# Autodesk Inventor assembly: base mg996r 3mm frame top
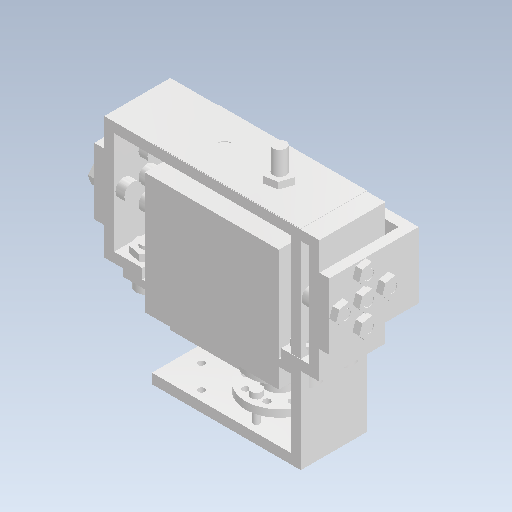
[picture p0: Inventor's stored thumbnail of the model, 512x512]
Saved by Autodesk Inventor 2021.4 (Build 254397000, 397)
## iProperties
Created: 2022-07-09
Part Number: base mg996r 3mm frame top
Document SubType Name: Assembly
Designer: isamu
Author: isamu
## Documents named in this file (5)
- D:\personal_projects\robot\inventor\2021\base mg996r 3mm frame top.iam
- D:\personal_projects\robot\exports\frames\servo frame part 3.ipt
- D:\personal_projects\robot\exports\screws\m3x8.ipt
- D:\personal_projects\robot\exports\screws\m3 nuts.ipt
- D:\personal_projects\robot\inventor\2021\base mg996r 3mm frame with axis.iam
## Components (22 placed, 4 different names)
1. servo frame part 3:1 — Mate:1, Mate:2, Mate:3, Insert:16, Insert:17, Insert:18, Insert:19, Insert:20, Insert:21, Insert:22, Insert:23, Insert:24, Insert:25
2. m3x8:1 — Insert:3
3. m3x8:2 — Insert:5
4. m3x8:3 — Insert:6
5. m3x8:4 — Insert:9
6. m3x8:5 — Insert:7
7. m3x8:6 — Insert:8
8. m3x8:7 — Insert:10
9. m3x8:9 — Insert:1
10. m3x8:11 — Insert:2
11. m3x8:12 — Insert:4
12. m3 nuts:1 — Insert:23
13. m3 nuts:2 — Insert:19
14. m3 nuts:3 — Insert:18
15. m3 nuts:4 — Insert:17
16. m3 nuts:5 — Insert:16
17. m3 nuts:6 — Insert:20
18. m3 nuts:7 — Insert:22
19. m3 nuts:8 — Insert:24
20. m3 nuts:9 — Insert:25
21. m3 nuts:10 — Insert:21
22. base mg996r 3mm frame with axis:1 [sub-assembly] — Mate:1, Mate:2, Mate:3, Insert:1, Insert:2, Insert:3, Insert:4, Insert:5, Insert:6, Insert:7, Insert:8, Insert:9, Insert:10
## Relationships (23: Insert 20, Mate 3)
- Mate:1: servo frame part 3:1 ↔ base mg996r 3mm frame with axis:1
- Mate:2: servo frame part 3:1 ↔ base mg996r 3mm frame with axis:1
- Mate:3: servo frame part 3:1 ↔ base mg996r 3mm frame with axis:1
- Insert:1: m3x8:9 ↔ base mg996r 3mm frame with axis:1
- Insert:2: m3x8:11 ↔ base mg996r 3mm frame with axis:1
- Insert:3: m3x8:1 ↔ base mg996r 3mm frame with axis:1
- Insert:4: m3x8:12 ↔ base mg996r 3mm frame with axis:1
- Insert:5: m3x8:2 ↔ base mg996r 3mm frame with axis:1
- Insert:6: m3x8:3 ↔ base mg996r 3mm frame with axis:1
- Insert:7: m3x8:5 ↔ base mg996r 3mm frame with axis:1
- Insert:8: m3x8:6 ↔ base mg996r 3mm frame with axis:1
- Insert:9: m3x8:4 ↔ base mg996r 3mm frame with axis:1
- Insert:10: m3x8:7 ↔ base mg996r 3mm frame with axis:1
- Insert:16: servo frame part 3:1 ↔ m3 nuts:5
- Insert:17: servo frame part 3:1 ↔ m3 nuts:4
- Insert:18: servo frame part 3:1 ↔ m3 nuts:3
- Insert:19: servo frame part 3:1 ↔ m3 nuts:2
- Insert:20: servo frame part 3:1 ↔ m3 nuts:6
- Insert:21: servo frame part 3:1 ↔ m3 nuts:10
- Insert:22: servo frame part 3:1 ↔ m3 nuts:7
- Insert:23: servo frame part 3:1 ↔ m3 nuts:1
- Insert:24: servo frame part 3:1 ↔ m3 nuts:8
- Insert:25: servo frame part 3:1 ↔ m3 nuts:9
